# Autodesk Inventor assembly: Robot
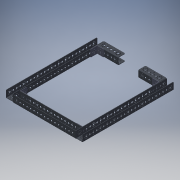
[picture p0: Inventor's stored thumbnail of the model, 180x180]
Saved by Autodesk Inventor 2016 (Build 200138000, 138)
## iProperties
Created: 2015-11-11
Part Number: Robot
Document SubType Name: Assembly
Designer: Julia
Author: Julia
## Documents named in this file (5)
- C:\Users\Julia\Documents\FTC CAD Parts\Robot.iam
- C:\Users\Julia\Documents\FTC CAD Parts\Tetrix_Kit_FTC\tetrix_739066_2012.ipt
- C:\Users\Julia\Documents\FTC CAD Parts\Tetrix_Kit_FTC\tetrix_739068_2012.ipt
- C:\Users\Julia\Documents\FTC CAD Parts\Tetrix_Kit_FTC\tetrix_739069_2012.ipt
- C:\Users\Julia\Documents\FTC CAD Parts\Tetrix_Kit_FTC\tetrix_739281_corner_bra_2013.ipt
## Components (9 placed, 4 different names)
1. tetrix_739066_2012:1 — Mate:11, Mate:12, Mate:18
2. tetrix_739066_2012:2 — Mate:13, Mate:14, Mate:16
3. tetrix_739068_2012:1 — Mate:1, Mate:2, Mate:3, Mate:4, Mate:5, Mate:6, Mate:8, Mate:10
4. tetrix_739069_2012:1 — Mate:1, Mate:2, Mate:3, Mate:7, Mate:13, Mate:14, Mate:15
5. tetrix_739069_2012:2 — Mate:4, Mate:5, Mate:6, Mate:9, Mate:11, Mate:12, Mate:17
6. tetrix_739281_corner_bra_2013:1 — Mate:9, Mate:10
7. tetrix_739281_corner_bra_2013:2 — Mate:17, Mate:18
8. tetrix_739281_corner_bra_2013:3 — Mate:7, Mate:8
9. tetrix_739281_corner_bra_2013:4 — Mate:15, Mate:16
## Relationships (18: Mate 18)
- Mate:1: tetrix_739068_2012:1 ↔ tetrix_739069_2012:1
- Mate:2: tetrix_739068_2012:1 ↔ tetrix_739069_2012:1
- Mate:3: tetrix_739068_2012:1 ↔ tetrix_739069_2012:1
- Mate:4: tetrix_739068_2012:1 ↔ tetrix_739069_2012:2
- Mate:5: tetrix_739068_2012:1 ↔ tetrix_739069_2012:2
- Mate:6: tetrix_739068_2012:1 ↔ tetrix_739069_2012:2
- Mate:7: tetrix_739069_2012:1 ↔ tetrix_739281_corner_bra_2013:3
- Mate:8: tetrix_739068_2012:1 ↔ tetrix_739281_corner_bra_2013:3
- Mate:9: tetrix_739069_2012:2 ↔ tetrix_739281_corner_bra_2013:1
- Mate:10: tetrix_739068_2012:1 ↔ tetrix_739281_corner_bra_2013:1
- Mate:11: tetrix_739066_2012:1 ↔ tetrix_739069_2012:2
- Mate:12: tetrix_739066_2012:1 ↔ tetrix_739069_2012:2
- Mate:13: tetrix_739066_2012:2 ↔ tetrix_739069_2012:1
- Mate:14: tetrix_739066_2012:2 ↔ tetrix_739069_2012:1
- Mate:15: tetrix_739069_2012:1 ↔ tetrix_739281_corner_bra_2013:4
- Mate:16: tetrix_739066_2012:2 ↔ tetrix_739281_corner_bra_2013:4
- Mate:17: tetrix_739069_2012:2 ↔ tetrix_739281_corner_bra_2013:2
- Mate:18: tetrix_739066_2012:1 ↔ tetrix_739281_corner_bra_2013:2
